# Autodesk Inventor assembly: suspension_one_side
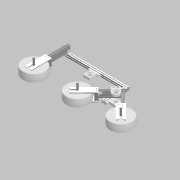
[picture p0: Inventor's stored thumbnail of the model, 180x180]
Saved by Autodesk Inventor 2021.2 (Build 252289000, 289)
## iProperties
Created: 2021-05-27
Part Number: suspension_one_side
Document SubType Name: Assembly
Designer: gisen
Author: gisen
## Documents named in this file (8)
- C:\Users\gisen\workspace\beetle_inventor_model\suspension\rocker_bogie_left.iam
- C:\Users\gisen\workspace\beetle_inventor_model\suspension\rocker.iam
- C:\Users\gisen\workspace\beetle_inventor_model\suspension\bogie.iam
- C:\Users\gisen\workspace\beetle_inventor_model\suspension\BSHKSA6904ZZ-40\BSHKSA6904ZZ-40.iam
- C:\Users\gisen\workspace\beetle_inventor_model\suspension\AFS-2020-4-430.ipt
- C:\Users\gisen\workspace\beetle_inventor_model\suspension\M4L.ipt
- C:\Users\gisen\workspace\beetle_inventor_model\suspension\AFS-2020-4-150.ipt
- C:\Users\gisen\workspace\beetle_inventor_model\suspension\rocker_bogie_mount.ipt
## Components (9 placed, 7 different names)
1. rocker:1 [sub-assembly] — メイト:1, フラッシュ:1, フラッシュ:2, メイト:3, 角度:1, メイト:11, メイト:13, メイト:14, メイト:18, 対称度:1
2. bogie:1 [sub-assembly] — フラッシュ:1, メイト:3, メイト:4, フラッシュ:3, メイト:6, メイト:9
3. AFS-2020-4-150:1 — メイト:5, メイト:7, フラッシュ:9, メイト:9, 角度:2, フラッシュ:4, フラッシュ:5, メイト:10
4. BSHKSA6904ZZ-40:1 [sub-assembly] — メイト:5, メイト:6, メイト:7, フラッシュ:9
5. AFS-2020-4-430:1 — フラッシュ:4, フラッシュ:5, メイト:10, メイト:12, メイト:15, フラッシュ:10, メイト:16, メイト:17, メイト:19, メイト:20, メイト:21, 対称度:1
6. M4L:1 — メイト:11, メイト:12, メイト:13
7. rocker_bogie_mount:1 — メイト:14, メイト:15, フラッシュ:10
8. M4L:2 — メイト:16, メイト:17, メイト:18
9. BSHKSA6904ZZ-40:2 [sub-assembly] — メイト:19, メイト:20, メイト:21, メイト:22
## Relationships (30: Mate 20, Flush 7, Angle 2, Symmetry 1)
- メイト:1 [Mate]: rocker:1
- フラッシュ:1 [Flush]: rocker:1 ↔ bogie:1
- フラッシュ:2 [Flush]: rocker:1
- メイト:3 [Mate] (300 mm): rocker:1 ↔ bogie:1
- メイト:4 [Mate]: bogie:1
- フラッシュ:3 [Flush]: bogie:1
- メイト:5 [Mate]: AFS-2020-4-150:1 ↔ BSHKSA6904ZZ-40:1
- メイト:6 [Mate]: bogie:1 ↔ BSHKSA6904ZZ-40:1
- メイト:7 [Mate] (-10 mm): AFS-2020-4-150:1 ↔ BSHKSA6904ZZ-40:1
- フラッシュ:9 [Flush]: AFS-2020-4-150:1 ↔ BSHKSA6904ZZ-40:1
- メイト:9 [Mate] (3 mm): bogie:1 ↔ AFS-2020-4-150:1
- 角度:1 [Angle] (180 deg): rocker:1
- 角度:2 [Angle] (180 deg): AFS-2020-4-150:1
- フラッシュ:4 [Flush]: AFS-2020-4-150:1 ↔ AFS-2020-4-430:1
- フラッシュ:5 [Flush]: AFS-2020-4-150:1 ↔ AFS-2020-4-430:1
- メイト:10 [Mate]: AFS-2020-4-150:1 ↔ AFS-2020-4-430:1
- メイト:11 [Mate]: rocker:1 ↔ M4L:1
- メイト:12 [Mate]: AFS-2020-4-430:1 ↔ M4L:1
- メイト:13 [Mate] (-10 mm): rocker:1 ↔ M4L:1
- メイト:14 [Mate]: rocker:1 ↔ rocker_bogie_mount:1
- メイト:15 [Mate]: AFS-2020-4-430:1 ↔ rocker_bogie_mount:1
- フラッシュ:10 [Flush]: AFS-2020-4-430:1 ↔ rocker_bogie_mount:1
- メイト:16 [Mate]: AFS-2020-4-430:1 ↔ M4L:2
- メイト:17 [Mate] (-10 mm): AFS-2020-4-430:1 ↔ M4L:2
- メイト:18 [Mate]: rocker:1 ↔ M4L:2
- メイト:19 [Mate]: AFS-2020-4-430:1 ↔ BSHKSA6904ZZ-40:2
- メイト:20 [Mate] (-10 mm): AFS-2020-4-430:1 ↔ BSHKSA6904ZZ-40:2
- メイト:21 [Mate] (-10 mm): AFS-2020-4-430:1 ↔ BSHKSA6904ZZ-40:2
- 対称度:1 [Symmetry]: rocker:1 ↔ AFS-2020-4-430:1
- メイト:22 [Mate]: BSHKSA6904ZZ-40:2
